# Autodesk Inventor assembly: new_ude
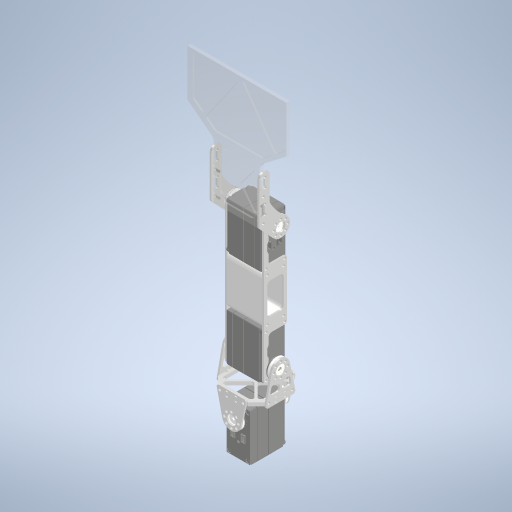
[picture p0: Inventor's stored thumbnail of the model, 512x512]
Saved by Autodesk Inventor 2024 (Build 280153000, 153)
## iProperties
Created: 2023-12-16
Part Number: new_ude
Document SubType Name: Assembly
Designer: right
Mass: 177.56 g
Surface Area: 658.267 cm^2
Volume: 114.096 cm^3
Density: 1.55623 g/cm^3
Author: right
## Documents named in this file (16)
- C:\Users\right\OneDrive\ドキュメント\Inventor\V2二足Light＿仮\new_ude.iam
- C:\Users\right\OneDrive\ドキュメント\Inventor\V2二足Light＿仮\KRS2500_scale3.ipt
- C:\Users\right\OneDrive\ドキュメント\Inventor\V2二足Light＿仮\02159_SmallFreeHornC_MIR2.ipt
- C:\Users\right\OneDrive\ドキュメント\Inventor\V2二足Light＿仮\02157_SmallDiameterHornB_MIR1.ipt
- C:\Users\right\OneDrive\ドキュメント\Inventor\V2二足Light＿仮\kata_new.ipt
- C:\Users\right\OneDrive\ドキュメント\Inventor\V2二足Light＿仮\new_kata_3.ipt
- C:\Users\right\OneDrive\ドキュメント\Inventor\V2二足Light＿仮\kata_new_1.5.ipt
- C:\Users\right\OneDrive\ドキュメント\Inventor\V2二足Light＿仮\new_ude.ipt
- C:\Users\right\OneDrive\ドキュメント\Inventor\V2二足Light＿仮\suzikai.ipt
- C:\Users\right\OneDrive\ドキュメント\Inventor\V2二足Light＿仮\Assembly_1.iam
- C:\Users\right\OneDrive\ドキュメント\Inventor\V2二足Light＿仮\new_ude\AIP\FEA\ejufw0veo.fins
- C:\Users\right\OneDrive\ドキュメント\Inventor\V2二足Light＿仮\new_ude\AIP\FEA\ejufw0veo.fsat
- C:\Users\right\OneDrive\ドキュメント\Inventor\V2二足Light＿仮\new_ude\AIP\FEA\ejufw0vfk.ftes
- C:\Users\right\OneDrive\ドキュメント\Inventor\V2二足Light＿仮\new_ude\AIP\FEA\ejufw0vfk.fwiz
- C:\Users\right\OneDrive\ドキュメント\Inventor\V2二足Light＿仮\new_ude\AIP\FEA\ejufw0w00.fmsh
- C:\Users\right\OneDrive\ドキュメント\Inventor\V2二足Light＿仮\new_ude\AIP\FEA\ejufw0w01.fres
## Components (18 placed, 9 different names)
1. KRS2500_scale3:1 — 挿入:1, 挿入:2, 角度:1
2. 02159_SmallFreeHornC_MIR2:1 — 挿入:1, 挿入:5, 挿入:6
3. 02157_SmallDiameterHornB_MIR1:1 — 挿入:2, フラッシュ:1, 挿入:3, 挿入:4
4. kata_new:1 — フラッシュ:1, 挿入:3, 挿入:4, フラッシュ:2, 挿入:8, 挿入:9
5. new_kata_3:1 — フラッシュ:2, 挿入:7, 挿入:8, 挿入:9, 挿入:10, 挿入:11, 挿入:12, 挿入:13, 挿入:14
6. kata_new:2 — 挿入:5, 挿入:6, 挿入:7, 挿入:10
7. kata_new_1.5:1 — 挿入:11, 挿入:12, 挿入:17, 挿入:18
8. kata_new_1.5:2 — 挿入:13, 挿入:14, 挿入:19, 挿入:20
9. KRS2500_scale3:2 — フラッシュ:4, 挿入:21, 挿入:22, 角度:1
10. 02159_SmallFreeHornC_MIR2:2 — 挿入:19, 挿入:20
11. 02157_SmallDiameterHornB_MIR1:2 — 挿入:17, 挿入:18
12. new_ude:1 — フラッシュ:4, 挿入:54
13. new_ude:2 — 挿入:21, 挿入:22, 挿入:51, 挿入:52, 挿入:53
14. KRS2500_scale3:3 — 挿入:49, 挿入:50, 挿入:51, 挿入:52
15. 02157_SmallDiameterHornB_MIR1:5 — 挿入:50, 挿入:55
16. 02159_SmallFreeHornC_MIR2:3 — 挿入:49, 挿入:56, 挿入:57
17. suzikai:1 — 挿入:53, 挿入:54
18. Assembly_1:1 [sub-assembly] — 挿入:55, 挿入:56, 挿入:57
## Relationships (35: Insert 31, Flush 3, Angle 1)
- 挿入:1 [Insert]: KRS2500_scale3:1 ↔ 02159_SmallFreeHornC_MIR2:1
- 挿入:2 [Insert]: KRS2500_scale3:1 ↔ 02157_SmallDiameterHornB_MIR1:1
- フラッシュ:1 [Flush]: 02157_SmallDiameterHornB_MIR1:1 ↔ kata_new:1
- 挿入:3 [Insert]: 02157_SmallDiameterHornB_MIR1:1 ↔ kata_new:1
- 挿入:4 [Insert]: 02157_SmallDiameterHornB_MIR1:1 ↔ kata_new:1
- フラッシュ:2 [Flush]: kata_new:1 ↔ new_kata_3:1
- 挿入:5 [Insert]: 02159_SmallFreeHornC_MIR2:1 ↔ kata_new:2
- 挿入:6 [Insert]: 02159_SmallFreeHornC_MIR2:1 ↔ kata_new:2
- 挿入:7 [Insert]: new_kata_3:1 ↔ kata_new:2
- 挿入:8 [Insert]: kata_new:1 ↔ new_kata_3:1
- 挿入:9 [Insert]: kata_new:1 ↔ new_kata_3:1
- 挿入:10 [Insert]: new_kata_3:1 ↔ kata_new:2
- 挿入:11 [Insert]: new_kata_3:1 ↔ kata_new_1.5:1
- 挿入:12 [Insert]: new_kata_3:1 ↔ kata_new_1.5:1
- 挿入:13 [Insert]: new_kata_3:1 ↔ kata_new_1.5:2
- 挿入:14 [Insert]: new_kata_3:1 ↔ kata_new_1.5:2
- [Insert]: KRS2500_scale3:2 ↔ 02159_SmallFreeHornC_MIR2:2
- [Insert]: KRS2500_scale3:2 ↔ 02157_SmallDiameterHornB_MIR1:2
- 挿入:17 [Insert]: kata_new_1.5:1 ↔ 02157_SmallDiameterHornB_MIR1:2
- 挿入:18 [Insert]: kata_new_1.5:1 ↔ 02157_SmallDiameterHornB_MIR1:2
- 挿入:19 [Insert]: kata_new_1.5:2 ↔ 02159_SmallFreeHornC_MIR2:2
- 挿入:20 [Insert]: kata_new_1.5:2 ↔ 02159_SmallFreeHornC_MIR2:2
- フラッシュ:4 [Flush]: KRS2500_scale3:2 ↔ new_ude:1
- 挿入:21 [Insert]: KRS2500_scale3:2 ↔ new_ude:2
- 挿入:22 [Insert]: KRS2500_scale3:2 ↔ new_ude:2
- 角度:1 [Angle] (0 deg): KRS2500_scale3:1 ↔ KRS2500_scale3:2
- 挿入:49 [Insert]: KRS2500_scale3:3 ↔ 02159_SmallFreeHornC_MIR2:3
- 挿入:50 [Insert]: KRS2500_scale3:3 ↔ 02157_SmallDiameterHornB_MIR1:5
- 挿入:51 [Insert]: new_ude:2 ↔ KRS2500_scale3:3
- 挿入:52 [Insert]: new_ude:2 ↔ KRS2500_scale3:3
- 挿入:53 [Insert]: new_ude:2 ↔ suzikai:1
- 挿入:54 [Insert]: new_ude:1 ↔ suzikai:1
- 挿入:55 [Insert]: 02157_SmallDiameterHornB_MIR1:5 ↔ Assembly_1:1
- 挿入:56 [Insert]: 02159_SmallFreeHornC_MIR2:3 ↔ Assembly_1:1
- 挿入:57 [Insert]: 02159_SmallFreeHornC_MIR2:3 ↔ Assembly_1:1
## Named parameters: d20_d1 = 0 mm, d21_d0 = 0 mm, sa_0 = 0, sa_1 = 0, sa_2 = -1176
note: some values were not read from the file. Shown as the stored number, unit unknown: "sa_0", "sa_1", "sa_2".
